# Autodesk Inventor assembly: 大锥齿轮-主动轮
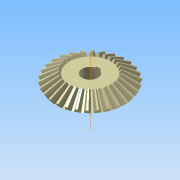
[picture p0: Inventor's stored thumbnail of the model, 180x180]
Saved by Autodesk Inventor 2015 (Build 190159000, 159)
## iProperties
Created: 2017-05-24
Part Number: 大锥齿轮-主动轮
Document SubType Name: Assembly
Designer: Administrator
Author: Administrator
## Documents named in this file (3)
- C:\Users\Administrator\Desktop\毕设改\中间传动大锥齿轮.iam
- C:\Users\Administrator\Desktop\毕设改\大锥齿轮-主动轮\设计加速器\大锥齿轮-主动轮2.iam
- C:\Users\Administrator\Desktop\毕设改\中间传动大锥齿轮配件.ipt
## Components (2 placed, 2 different names)
1. 大锥齿轮-主动轮:1 [sub-assembly] — 插入:1, 表面齐平:1
2. 中间传动大锥齿轮配件:1 — 插入:1, 表面齐平:1
## Relationships (2: Insert 1, Flush 1)
- 插入:1 [Insert]: 大锥齿轮-主动轮:1 ↔ 中间传动大锥齿轮配件:1
- 表面齐平:1 [Flush]: 大锥齿轮-主动轮:1 ↔ 中间传动大锥齿轮配件:1
